# Autodesk Inventor assembly: HUB TOP
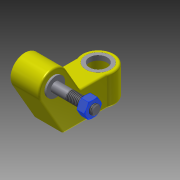
[picture p0: Inventor's stored thumbnail of the model, 180x180]
Saved by Autodesk Inventor 2013 (Build 170138000, 138)
## iProperties
Created: 2013-11-27
Part Number: HUB TOP
Document SubType Name: Assembly
Designer: employee
Author: employee
## Documents named in this file (6)
- C:\Users\employee\Desktop\GUS Simpson\HUB TOP.iam
- C:\Users\employee\Desktop\GUS Simpson\HUB TOP.ipt
- C:\Users\employee\Desktop\GUS Simpson\_6702.ipt
- C:\Users\employee\Desktop\GUS Simpson\M8x55.ipt
- C:\Users\employee\Desktop\GUS Simpson\M8 WASHER.ipt
- C:\Users\employee\Desktop\GUS Simpson\M8 NUT.ipt
## Components (6 placed, 5 different names)
1. HUB TOP:1 — Insert:1, Insert:2, Insert:3, Angle:1, Insert:4, Angle:2
2. _6702:1 — Insert:1
3. _6702:2 — Insert:2
4. M8x55:1 — Insert:3, Angle:1
5. M8 WASHER:1 — Insert:4, Insert:5
6. M8 NUT:1 — Insert:5, Angle:2
## Relationships (7: Insert 5, Angle 2)
- Insert:1: HUB TOP:1 ↔ _6702:1
- Insert:2: HUB TOP:1 ↔ _6702:2
- Insert:3: HUB TOP:1 ↔ M8x55:1
- Angle:1 (0 deg): HUB TOP:1 ↔ M8x55:1
- Insert:4: HUB TOP:1 ↔ M8 WASHER:1
- Insert:5 (25 mm): M8 WASHER:1 ↔ M8 NUT:1
- Angle:2 (0 deg): HUB TOP:1 ↔ M8 NUT:1
